# Autodesk Inventor assembly: A1-18002-200-00 Skid leg
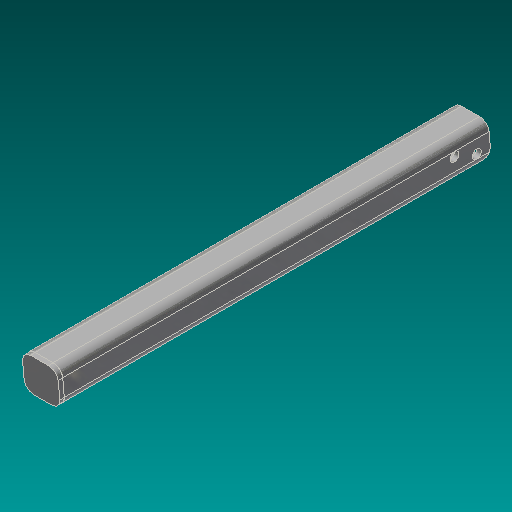
[picture p0: Inventor's stored thumbnail of the model, 512x512]
Saved by Autodesk Inventor 2017 (Build 210142000, 142)
## iProperties
Created: 2018-01-24
Part Number: A1-18002-200-00 Skid leg
Document SubType Name: Assembly
Designer: Graeme_Van_Dongen
Author: Graeme_Van_Dongen
## Documents named in this file (3)
- N:\A1 - Projects\A1-18\A1-18002--Alco Line boring skid\A1-18002-200-00 Skid leg.iam
- N:\A1 - Projects\A1-18\A1-18002--Alco Line boring skid\A1-18002-200-01 Leg tube.ipt
- N:\A1 - Projects\A1-18\A1-18002--Alco Line boring skid\A1-18002-200-02 Foot plate.ipt
## Components (2 placed, 2 different names)
1. A1-18002-200-01 Leg tube:1 — Mate:1, Mate:2, Flush:2
2. A1-18002-200-02 Foot plate:1 — Mate:1, Mate:2, Flush:2
## Relationships (3: Mate 2, Flush 1)
- Mate:1: A1-18002-200-01 Leg tube:1 ↔ A1-18002-200-02 Foot plate:1
- Mate:2: A1-18002-200-01 Leg tube:1 ↔ A1-18002-200-02 Foot plate:1
- Flush:2: A1-18002-200-01 Leg tube:1 ↔ A1-18002-200-02 Foot plate:1
